# Autodesk Inventor assembly: ensamble_general
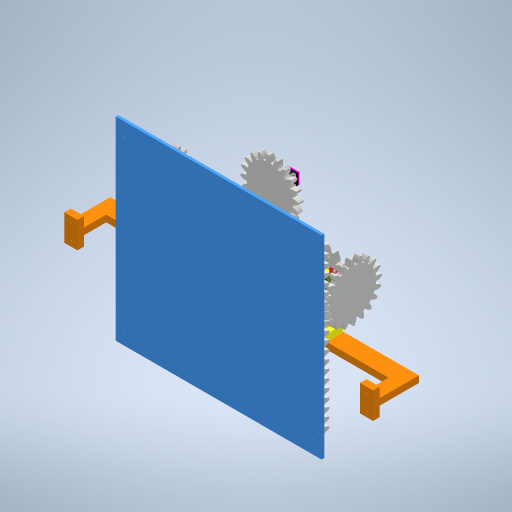
[picture p0: Inventor's stored thumbnail of the model, 512x512]
Saved by Autodesk Inventor 2023.2 (Build 272271030, 271C)
## iProperties
Created: 2023-03-04
Part Number: ensamble_general
Document SubType Name: Assembly
Designer: Cris Pat
Author: Cris Pat
## Documents named in this file (20)
- C:\Users\Cris Pat\Desktop\U\Semestre 9\disenio e innovacion\CAD\Impresion 3D\robotH\ensamble_general.iam
- C:\Users\Cris Pat\Desktop\U\Semestre 9\disenio e innovacion\CAD\Impresion 3D\robotH\eje.iam
- C:\Users\Cris Pat\Desktop\U\Semestre 9\disenio e innovacion\CAD\Impresion 3D\robotH\piñon1.ipt
- C:\Users\Cris Pat\Desktop\U\Semestre 9\disenio e innovacion\CAD\Impresion 3D\robotH\stepper.ipt
- C:\Users\Cris Pat\Desktop\U\Semestre 9\disenio e innovacion\CAD\Impresion 3D\robotH\eje steper.ipt
- C:\Users\Cris Pat\Desktop\U\Semestre 9\disenio e innovacion\CAD\Impresion 3D\robotH\sostenedor.iam
- C:\Users\Cris Pat\Desktop\U\Semestre 9\disenio e innovacion\CAD\Impresion 3D\robotH\cremallera1.ipt
- C:\Users\Cris Pat\Desktop\U\Semestre 9\disenio e innovacion\CAD\Impresion 3D\robotH\libreria\en-US\DIN 84\DIN 84 - M5 x 28.ipt
- C:\Users\Cris Pat\Desktop\U\Semestre 9\disenio e innovacion\CAD\Impresion 3D\robotH\libreria\en-US\DIN 439-2\DIN 439 - M5 x 0.8.ipt
- C:\Users\Cris Pat\Desktop\U\Semestre 9\disenio e innovacion\CAD\Impresion 3D\robotH\lamina.ipt
- C:\Users\Cris Pat\Desktop\U\Semestre 9\disenio e innovacion\CAD\Impresion 3D\robotH\sostenedor_part1.ipt
- C:\Users\Cris Pat\Desktop\U\Semestre 9\disenio e innovacion\CAD\Impresion 3D\robotH\detenedor.ipt
- C:\Users\Cris Pat\Desktop\U\Semestre 9\disenio e innovacion\CAD\Impresion 3D\robotH\patas.ipt
- C:\Users\Cris Pat\Desktop\U\Semestre 9\disenio e innovacion\CAD\Impresion 3D\robotH\libreria\en-US\DIN 84\DIN 84 - M5 x 50.ipt
- C:\Users\Cris Pat\Desktop\U\Semestre 9\disenio e innovacion\CAD\Impresion 3D\robotH\libreria\en-US\DIN 84\DIN 84 - M5 x 25.ipt
- C:\Users\Cris Pat\Desktop\U\Semestre 9\disenio e innovacion\CAD\Impresion 3D\robotH\libreria\en-US\DIN 84\DIN 84 - M5 x 22.ipt
- C:\Users\Cris Pat\Desktop\U\Semestre 9\disenio e innovacion\CAD\Impresion 3D\robotH\libreria\en-US\DIN 84\DIN 84 - M5 x 10.ipt
- C:\Users\Cris Pat\Desktop\U\Semestre 9\disenio e innovacion\CAD\Impresion 3D\robotH\libreria\en-US\DIN 84\DIN 84 - M8 x 14.ipt
- C:\Users\Cris Pat\Desktop\U\Semestre 9\disenio e innovacion\CAD\Impresion 3D\robotH\patas2.ipt
- C:\Users\Cris Pat\Desktop\U\Semestre 9\disenio e innovacion\CAD\Impresion 3D\robotH\libreria\en-US\DIN 84\DIN 84 - M5 x 50A.ipt
## Components (78 placed, 18 different names)
1. eje:1 [sub-assembly] — Flush:1, Flush:2, Mate:2, Rotation/Translation:1, Flush:4, Mate:4, Mate:5, Flush:8, Mate:13, Mate:14, Mate:17, Mate:18
2. piñon1:1 — Flush:1, Rigid:1, Flush:2, Rotation/Translation:1
3. stepper:1 — Rotational:1, Mate:1, Angle:1, Flush:9, Insert:25, Insert:26, Insert:27, Insert:28
4. eje steper:1 — Rotational:1, Rigid:1
5. stepper:2 — Mate:3, Rigid:2, Rigid:3, Rotational:2, Insert:7, Insert:8, Mate:22, Flush:11, Mate:23, Insert:37, Insert:38
6. sostenedor:1 [sub-assembly] — Mate:3, Rigid:2, Insert:11, Insert:14
7. sostenedor:2 [sub-assembly] — Rigid:3, Flush:4, Mate:4, Mate:5, Insert:12, Insert:13
8. eje steper:2 — Rotational:2, Rigid:4
9. piñon1:2 — Rigid:4, Flush:7, Rotation/Translation:2
10. cremallera1:1 — Flush:7, Mate:12, Rotation/Translation:2, Rigid:5, Insert:54, Insert:55
11. DIN 84 - replaced by DIN EN ISO 1207 M5 x 28:1 — Insert:7
12. DIN 84 - replaced by DIN EN ISO 1207 M5 x 28:2 — Insert:8
13. DIN 439-2 - replaced by DIN EN 24035/28675 M5:1 — Insert:11
14. DIN 439-2 - replaced by DIN EN 24035/28675 M5:2 — Insert:12
15. DIN 439-2 - replaced by DIN EN 24035/28675 M5:3 — Insert:13
16. DIN 439-2 - replaced by DIN EN 24035/28675 M5:4 — Insert:14
17. lamina:1 — Rigid:5, Rigid:6
18. cremallera1:2 — Rigid:6, Rotation/Translation:3, Insert:52, Insert:53
19. stepper:3 — Rotational:3, Rigid:7, Rigid:8, Mate:20, Flush:10, Mate:21, Insert:16, Insert:20, Insert:39, Insert:41
20. eje steper:3 — Rotational:3, Rotational:4
21. sostenedor:3 [sub-assembly] — Rigid:7, Mate:15, Insert:15, Insert:18
22. sostenedor:4 [sub-assembly] — Rigid:8, Flush:8, Mate:13, Mate:14, Mate:16, Insert:17, Insert:19
23. DIN 439-2 - replaced by DIN EN 24035/28675 M5:5 — Mate:15
24. DIN 439-2 - replaced by DIN EN 24035/28675 M5:6 — Mate:16
25. piñon1:3 — Rotational:4, Rotation/Translation:3
26. sostenedor_part1:1 — Mate:17, Mate:18, Mate:19
27. detenedor:1 — Flush:9, Mate:19, Insert:47, Insert:48, Insert:49, Insert:50, Insert:51
28. patas:2 — Mate:20, Flush:10, Mate:21, Insert:29, Insert:30, Insert:31, Insert:32, Insert:43, Insert:44, Insert:45, Insert:46, Mate:24, Flush:13, Mate:25
29. patas:3 — Mate:22, Flush:11, Mate:23, Insert:21, Insert:22, Insert:23, Insert:24, Insert:33, Insert:34, Insert:35, Insert:36, Rigid:9
30. DIN 439-2 - replaced by DIN EN 24035/28675 M5:7 — Insert:15
31. DIN 439-2 - replaced by DIN EN 24035/28675 M5:8 — Insert:16
32. DIN 439-2 - replaced by DIN EN 24035/28675 M5:9 — Insert:17
33. DIN 439-2 - replaced by DIN EN 24035/28675 M5:10 — Insert:18
34. DIN 439-2 - replaced by DIN EN 24035/28675 M5:11 — Insert:19
35. DIN 439-2 - replaced by DIN EN 24035/28675 M5:12 — Insert:20
36. DIN 439-2 - replaced by DIN EN 24035/28675 M5:13 — Insert:21
37. DIN 439-2 - replaced by DIN EN 24035/28675 M5:14 — Insert:22
38. DIN 439-2 - replaced by DIN EN 24035/28675 M5:15 — Insert:23
39. DIN 439-2 - replaced by DIN EN 24035/28675 M5:16 — Insert:24
40. DIN 439-2 - replaced by DIN EN 24035/28675 M5:17 — Insert:25
41. DIN 439-2 - replaced by DIN EN 24035/28675 M5:18 — Insert:26
42. DIN 439-2 - replaced by DIN EN 24035/28675 M5:19 — Insert:27
43. DIN 439-2 - replaced by DIN EN 24035/28675 M5:20 — Insert:28
44. DIN 439-2 - replaced by DIN EN 24035/28675 M5:21 — Insert:29
45. DIN 439-2 - replaced by DIN EN 24035/28675 M5:22 — Insert:30
46. DIN 439-2 - replaced by DIN EN 24035/28675 M5:23 — Insert:31
47. DIN 439-2 - replaced by DIN EN 24035/28675 M5:24 — Insert:32
48. DIN 84 - replaced by DIN EN ISO 1207 M5 x 50:1 — Insert:33
49. DIN 84 - replaced by DIN EN ISO 1207 M5 x 50:2 — Insert:34
50. DIN 84 - replaced by DIN EN ISO 1207 M5 x 50:3 — Insert:35
51. DIN 84 - replaced by DIN EN ISO 1207 M5 x 50:4 — Insert:36
52. DIN 439-2 - replaced by DIN EN 24035/28675 M5:25 — Insert:37
53. DIN 439-2 - replaced by DIN EN 24035/28675 M5:26 — Insert:38
54. DIN 84 - replaced by DIN EN ISO 1207 M5 x 25:1 — Insert:39
55. DIN 84 - replaced by DIN EN ISO 1207 M5 x 25:3 — Insert:41
56. DIN 84 - replaced by DIN EN ISO 1207 M5 x 50:5 — Insert:43
57. DIN 84 - replaced by DIN EN ISO 1207 M5 x 50:6 — Insert:44
58. DIN 84 - replaced by DIN EN ISO 1207 M5 x 50:7 — Insert:45
59. DIN 84 - replaced by DIN EN ISO 1207 M5 x 50:8 — Insert:46
60. DIN 84 - replaced by DIN EN ISO 1207 M5 x 22:1 — Insert:47
61. DIN 84 - replaced by DIN EN ISO 1207 M5 x 22:2 — Insert:48
62. DIN 84 - replaced by DIN EN ISO 1207 M5 x 22:3 — Insert:49
63. DIN 84 - replaced by DIN EN ISO 1207 M5 x 22:4 — Insert:50
64. DIN 84 - replaced by DIN EN ISO 1207 M5 x 10:1 — Insert:51
65. DIN 84 - replaced by DIN EN ISO 1207 M8 x 14:1 — Insert:52
66. DIN 84 - replaced by DIN EN ISO 1207 M8 x 14:2 — Insert:53
67. DIN 84 - replaced by DIN EN ISO 1207 M8 x 14:3 — Insert:54
68. DIN 84 - replaced by DIN EN ISO 1207 M8 x 14:4 — Insert:55
69. patas2:2 — Mate:24, Flush:13, Mate:25, Insert:60, Insert:61, Insert:62, Insert:63
70. DIN 84 - replaced by DIN EN ISO 1207 M5 x 50:13 — Insert:60
71. DIN 84 - replaced by DIN EN ISO 1207 M5 x 50:18 — Insert:61
72. DIN 84 - replaced by DIN EN ISO 1207 M5 x 50:15 — Insert:62
73. DIN 84 - replaced by DIN EN ISO 1207 M5 x 50:16 — Insert:63
74. patas2:3 — Rigid:9, Insert:64, Insert:65, Insert:66, Insert:67
75. DIN 84 - replaced by DIN EN ISO 1207 M5 x 50:17 — Insert:64
76. DIN 84 - replaced by DIN EN ISO 1207 M5 x 50:19 — Insert:65
77. DIN 84 - replaced by DIN EN ISO 1207 M5 x 50:20 — Insert:66
78. DIN 84 - replaced by DIN EN ISO 1207 M5 x 50:21 — Insert:67
## Relationships (101: Insert 53, Mate 19, Flush 12, WeldJoint 9, RevoluteJoint 4, RelateRotateTranslate 3, Angle 1)
- Flush:1: eje:1 ↔ piñon1:1
- Rotational:1 [RevoluteJoint]: stepper:1 ↔ eje steper:1
- Rigid:1 [WeldJoint]: piñon1:1 ↔ eje steper:1
- Flush:2: eje:1 ↔ piñon1:1
- Mate:1: stepper:1
- Angle:1 (0 deg): stepper:1
- Flush:3 (100 mm)
- Mate:2 (12.5 mm): eje:1
- Rotation/Translation:1 [RelateRotateTranslate] (628.32 mm): eje:1 ↔ piñon1:1
- Mate:3: stepper:2 ↔ sostenedor:1
- Rigid:2 [WeldJoint]: stepper:2 ↔ sostenedor:1
- Rigid:3 [WeldJoint]: stepper:2 ↔ sostenedor:2
- Flush:4: eje:1 ↔ sostenedor:2
- Mate:4: eje:1 ↔ sostenedor:2
- Mate:5: eje:1 ↔ sostenedor:2
- Rotational:2 [RevoluteJoint]: stepper:2 ↔ eje steper:2
- Rigid:4 [WeldJoint]: eje steper:2 ↔ piñon1:2
- Flush:5 (-147.25 mm)
- Flush:6 (100 mm)
- Flush:7: piñon1:2 ↔ cremallera1:1
- Mate:12 (12.5 mm): cremallera1:1
- Rotation/Translation:2 [RelateRotateTranslate] (628.32 mm): piñon1:2 ↔ cremallera1:1
- Insert:7: stepper:2 ↔ DIN 84 - replaced by DIN EN ISO 1207 M5 x 28:1
- Insert:8: stepper:2 ↔ DIN 84 - replaced by DIN EN ISO 1207 M5 x 28:2
- Insert:11: sostenedor:1 ↔ DIN 439-2 - replaced by DIN EN 24035/28675 M5:1
- Insert:12: sostenedor:2 ↔ DIN 439-2 - replaced by DIN EN 24035/28675 M5:2
- Insert:13: sostenedor:2 ↔ DIN 439-2 - replaced by DIN EN 24035/28675 M5:3
- Insert:14: sostenedor:1 ↔ DIN 439-2 - replaced by DIN EN 24035/28675 M5:4
- Rigid:5 [WeldJoint]: cremallera1:1 ↔ lamina:1
- Rigid:6 [WeldJoint]: lamina:1 ↔ cremallera1:2
- Rotational:3 [RevoluteJoint]: stepper:3 ↔ eje steper:3
- Rigid:7 [WeldJoint]: stepper:3 ↔ sostenedor:3
- Rigid:8 [WeldJoint]: stepper:3 ↔ sostenedor:4
- Flush:8: eje:1 ↔ sostenedor:4
- Mate:13: eje:1 ↔ sostenedor:4
- Mate:14: eje:1 ↔ sostenedor:4
- Mate:15: sostenedor:3 ↔ DIN 439-2 - replaced by DIN EN 24035/28675 M5:5
- Mate:16: sostenedor:4 ↔ DIN 439-2 - replaced by DIN EN 24035/28675 M5:6
- Rotational:4 [RevoluteJoint]: eje steper:3 ↔ piñon1:3
- Rotation/Translation:3 [RelateRotateTranslate] (628.32 mm): cremallera1:2 ↔ piñon1:3
- Mate:17: eje:1 ↔ sostenedor_part1:1
- Mate:18: eje:1 ↔ sostenedor_part1:1
- Flush:9: stepper:1 ↔ detenedor:1
- Mate:19: sostenedor_part1:1 ↔ detenedor:1
- Mate:20: stepper:3 ↔ patas:2
- Flush:10: stepper:3 ↔ patas:2
- Mate:21: stepper:3 ↔ patas:2
- Mate:22: stepper:2 ↔ patas:3
- Flush:11: stepper:2 ↔ patas:3
- Mate:23: stepper:2 ↔ patas:3
- Insert:15: sostenedor:3 ↔ DIN 439-2 - replaced by DIN EN 24035/28675 M5:7
- Insert:16: stepper:3 ↔ DIN 439-2 - replaced by DIN EN 24035/28675 M5:8
- Insert:17: sostenedor:4 ↔ DIN 439-2 - replaced by DIN EN 24035/28675 M5:9
- Insert:18: sostenedor:3 ↔ DIN 439-2 - replaced by DIN EN 24035/28675 M5:10
- Insert:19: sostenedor:4 ↔ DIN 439-2 - replaced by DIN EN 24035/28675 M5:11
- Insert:20: stepper:3 ↔ DIN 439-2 - replaced by DIN EN 24035/28675 M5:12
- Insert:21: patas:3 ↔ DIN 439-2 - replaced by DIN EN 24035/28675 M5:13
- Insert:22: patas:3 ↔ DIN 439-2 - replaced by DIN EN 24035/28675 M5:14
- Insert:23: patas:3 ↔ DIN 439-2 - replaced by DIN EN 24035/28675 M5:15
- Insert:24: patas:3 ↔ DIN 439-2 - replaced by DIN EN 24035/28675 M5:16
- Insert:25: stepper:1 ↔ DIN 439-2 - replaced by DIN EN 24035/28675 M5:17
- Insert:26: stepper:1 ↔ DIN 439-2 - replaced by DIN EN 24035/28675 M5:18
- Insert:27: stepper:1 ↔ DIN 439-2 - replaced by DIN EN 24035/28675 M5:19
- Insert:28: stepper:1 ↔ DIN 439-2 - replaced by DIN EN 24035/28675 M5:20
- Insert:29: patas:2 ↔ DIN 439-2 - replaced by DIN EN 24035/28675 M5:21
- Insert:30: patas:2 ↔ DIN 439-2 - replaced by DIN EN 24035/28675 M5:22
- Insert:31: patas:2 ↔ DIN 439-2 - replaced by DIN EN 24035/28675 M5:23
- Insert:32: patas:2 ↔ DIN 439-2 - replaced by DIN EN 24035/28675 M5:24
- Insert:33: patas:3 ↔ DIN 84 - replaced by DIN EN ISO 1207 M5 x 50:1
- Insert:34: patas:3 ↔ DIN 84 - replaced by DIN EN ISO 1207 M5 x 50:2
- Insert:35: patas:3 ↔ DIN 84 - replaced by DIN EN ISO 1207 M5 x 50:3
- Insert:36: patas:3 ↔ DIN 84 - replaced by DIN EN ISO 1207 M5 x 50:4
- Insert:37: stepper:2 ↔ DIN 439-2 - replaced by DIN EN 24035/28675 M5:25
- Insert:38: stepper:2 ↔ DIN 439-2 - replaced by DIN EN 24035/28675 M5:26
- Insert:39: stepper:3 ↔ DIN 84 - replaced by DIN EN ISO 1207 M5 x 25:1
- Insert:41: stepper:3 ↔ DIN 84 - replaced by DIN EN ISO 1207 M5 x 25:3
- Insert:43: patas:2 ↔ DIN 84 - replaced by DIN EN ISO 1207 M5 x 50:5
- Insert:44: patas:2 ↔ DIN 84 - replaced by DIN EN ISO 1207 M5 x 50:6
- Insert:45: patas:2 ↔ DIN 84 - replaced by DIN EN ISO 1207 M5 x 50:7
- Insert:46: patas:2 ↔ DIN 84 - replaced by DIN EN ISO 1207 M5 x 50:8
- Insert:47: detenedor:1 ↔ DIN 84 - replaced by DIN EN ISO 1207 M5 x 22:1
- Insert:48: detenedor:1 ↔ DIN 84 - replaced by DIN EN ISO 1207 M5 x 22:2
- Insert:49: detenedor:1 ↔ DIN 84 - replaced by DIN EN ISO 1207 M5 x 22:3
- Insert:50: detenedor:1 ↔ DIN 84 - replaced by DIN EN ISO 1207 M5 x 22:4
- Insert:51: detenedor:1 ↔ DIN 84 - replaced by DIN EN ISO 1207 M5 x 10:1
- Insert:52: cremallera1:2 ↔ DIN 84 - replaced by DIN EN ISO 1207 M8 x 14:1
- Insert:53: cremallera1:2 ↔ DIN 84 - replaced by DIN EN ISO 1207 M8 x 14:2
- Insert:54: cremallera1:1 ↔ DIN 84 - replaced by DIN EN ISO 1207 M8 x 14:3
- Insert:55: cremallera1:1 ↔ DIN 84 - replaced by DIN EN ISO 1207 M8 x 14:4
- Mate:24: patas:2 ↔ patas2:2
- Flush:13: patas:2 ↔ patas2:2
- Mate:25: patas:2 ↔ patas2:2
- Insert:60: patas2:2 ↔ DIN 84 - replaced by DIN EN ISO 1207 M5 x 50:13
- Insert:61: patas2:2 ↔ DIN 84 - replaced by DIN EN ISO 1207 M5 x 50:18
- Insert:62: patas2:2 ↔ DIN 84 - replaced by DIN EN ISO 1207 M5 x 50:15
- Insert:63: patas2:2 ↔ DIN 84 - replaced by DIN EN ISO 1207 M5 x 50:16
- Rigid:9 [WeldJoint]: patas:3 ↔ patas2:3
- Insert:64: patas2:3 ↔ DIN 84 - replaced by DIN EN ISO 1207 M5 x 50:17
- Insert:65: patas2:3 ↔ DIN 84 - replaced by DIN EN ISO 1207 M5 x 50:19
- Insert:66: patas2:3 ↔ DIN 84 - replaced by DIN EN ISO 1207 M5 x 50:20
- Insert:67: patas2:3 ↔ DIN 84 - replaced by DIN EN ISO 1207 M5 x 50:21
